# Autodesk Inventor assembly: GP5-100
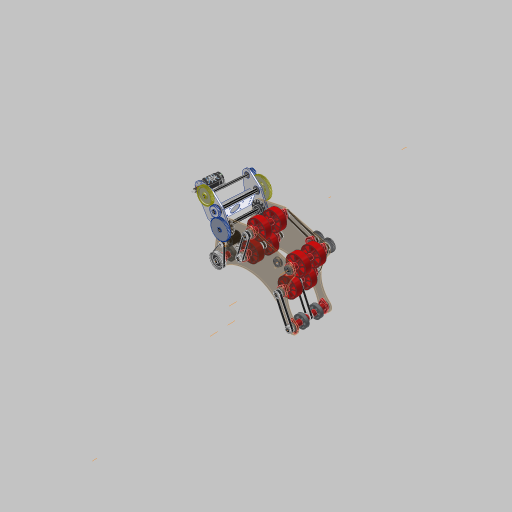
[picture p0: Inventor's stored thumbnail of the model, 512x512]
Saved by Autodesk Inventor 2023.5 (Build 275446000, 446)
## iProperties
Created: 2025-02-03
Part Number: GP5-100
Document SubType Name: Assembly
Designer: slick
Author: slick
## Documents named in this file (27)
- C:\Users\slick\OneDrive\Desktop\2025-ReefScape---CAD\Gripper\GP5\GP5-100.iam
- C:\Users\slick\OneDrive\Desktop\2025-ReefScape---CAD\Gripper\GP5\GP5-003.ipt
- C:\Users\slick\OneDrive\Desktop\2025-ReefScape---CAD\COMMON PARTS\BEARINGS\13_75mm_1_2_ThunderHex_ID_x_1_125_OD_x_0_313_WD_Flanged_Bearing_217-4006_MIR.ipt
- C:\Users\slick\OneDrive\Desktop\2025-ReefScape---CAD\Gripper\GP5\GP5-005.ipt
- C:\Users\slick\OneDrive\Desktop\2025-ReefScape---CAD\COMMON PARTS\WHEELS\2_OD_Straight_Flex_Wheel_217-6354.ipt
- C:\Users\slick\OneDrive\Desktop\2025-ReefScape---CAD\COMMON PARTS\WHEELS\am-3946 3IN 375Hex Compliant Wheel REV 3.ipt
- C:\Users\slick\OneDrive\Desktop\2025-ReefScape---CAD\COMMON PARTS\MOTORS\Minion.ipt
- C:\Users\slick\OneDrive\Desktop\2025-ReefScape---CAD\COMMON PARTS\PULLEYS\gt2\16T Gt2 Kracken PullyWCP-1178.ipt
- C:\Users\slick\OneDrive\Desktop\2025-ReefScape---CAD\COMMON PARTS\PULLEYS\gt2\60t_x_9mm_Wide_Double_Flange_Aluminum_Pulley_GT2_3mm_1_2_Hex_Bore_217-5876.ipt
- C:\Users\slick\OneDrive\Desktop\2025-ReefScape---CAD\COMMON PARTS\PULLEYS\gt2\24t_x_9mm_Wide_Double_Flange_Aluminum_Pulley_GT2_3mm_1_2_Hex_Bore_217-5875.ipt
- C:\Users\slick\OneDrive\Desktop\2025-ReefScape---CAD\COMMON PARTS\GEARS\20dp .5 hex\34t_Aluminum_Spur_Gear_20_DP_1_2_Hex_Bore_217-2706.ipt
- C:\Users\slick\OneDrive\Desktop\2025-ReefScape---CAD\Gripper\GP5\GP5-006.ipt
- C:\Users\slick\OneDrive\Desktop\2025-ReefScape---CAD\Gripper\GP5\GP5-007.ipt
- C:\Users\slick\OneDrive\Desktop\2025-ReefScape---CAD\Gripper\GP5\GP5-200.iam
- C:\Users\slick\OneDrive\Desktop\2025-ReefScape---CAD\COMMON PARTS\BEARINGS\Bearing Retainer\Retainer.ipt
- C:\Users\slick\OneDrive\Desktop\2025-ReefScape---CAD\Gripper\GP5\GT2-100T.ipt
- C:\Users\slick\OneDrive\Desktop\2025-ReefScape---CAD\Gripper\GP5\GT2-90T.ipt
- C:\Users\slick\OneDrive\Desktop\2025-ReefScape---CAD\Gripper\GP5\GT2-90T16-60.ipt
- C:\Users\slick\OneDrive\Desktop\2025-ReefScape---CAD\Gripper\GP5\GT2-105T.ipt
- C:\Users\slick\OneDrive\Desktop\2025-ReefScape---CAD\Gripper\GP5\GP5-013.ipt
- C:\Users\slick\OneDrive\Desktop\2025-ReefScape---CAD\Gripper\GP5\GP5-014.ipt
- C:\Users\slick\OneDrive\Desktop\2025-ReefScape---CAD\Gripper\GP5\GP5-015.ipt
- C:\Users\slick\OneDrive\Desktop\2025-ReefScape---CAD\Gripper\GP5\GP5-016.ipt
- C:\Users\slick\OneDrive\Desktop\2025-ReefScape---CAD\Gripper\GP5\GP5-017.ipt
- C:\Users\slick\OneDrive\Desktop\2025-ReefScape---CAD\Gripper\GP5\GP5-018.ipt
- C:\Users\slick\OneDrive\Desktop\2025-ReefScape---CAD\Gripper\GP5\GP5-019.ipt
- C:\Users\slick\OneDrive\Desktop\2025-ReefScape---CAD\COMMON PARTS\HUBS\WCP-1388.ipt
## Components (102 placed, 26 different names)
1. GP5-003:1 — Mate:7, Mate:9, Insert:12, Insert:13, Insert:14, Insert:15, Insert:16, Insert:17, Insert:18, Mate:49, Mate:59, Insert:21, Mate:64, Insert:22, Insert:23, Insert:24, Insert:25, Insert:26, Insert:27, Insert:28, Insert:29, Insert:30, Insert:31, Insert:32, Insert:33, Insert:34, Insert:35, Mate:137, Insert:49
2. GP5-003:2 — Mate:7, Mate:9, Insert:5, Insert:6, Insert:7, Insert:8, Insert:9, Insert:10, Insert:11, Mate:40, Mate:43, Mate:44, Insert:19, Mate:47, Mate:63, Insert:20, Insert:36, Insert:37, Insert:38, Insert:39, Insert:40, Insert:41, Insert:42, Insert:43, Insert:44, Insert:45, Insert:46, Insert:47, Mate:136, Insert:48
3. 13_75mm_1_2_ThunderHex_ID_x_1_125_OD_x_0_313_WD_Flanged_Bearing_217-4006_MIR:1 — Insert:5, Mate:20, Mate:46
4. 13_75mm_1_2_ThunderHex_ID_x_1_125_OD_x_0_313_WD_Flanged_Bearing_217-4006_MIR:2 — Insert:7, Mate:22
5. 13_75mm_1_2_ThunderHex_ID_x_1_125_OD_x_0_313_WD_Flanged_Bearing_217-4006_MIR:3 — Insert:6, Mate:21
6. 13_75mm_1_2_ThunderHex_ID_x_1_125_OD_x_0_313_WD_Flanged_Bearing_217-4006_MIR:4 — Insert:10, Mate:23, Mate:35, Mate:94
7. 13_75mm_1_2_ThunderHex_ID_x_1_125_OD_x_0_313_WD_Flanged_Bearing_217-4006_MIR:5 — Insert:9
8. 13_75mm_1_2_ThunderHex_ID_x_1_125_OD_x_0_313_WD_Flanged_Bearing_217-4006_MIR:6 — Insert:11, Mate:25
9. 13_75mm_1_2_ThunderHex_ID_x_1_125_OD_x_0_313_WD_Flanged_Bearing_217-4006_MIR:7 — Insert:8, Mate:24
10. 13_75mm_1_2_ThunderHex_ID_x_1_125_OD_x_0_313_WD_Flanged_Bearing_217-4006_MIR:8 — Insert:12
11. 13_75mm_1_2_ThunderHex_ID_x_1_125_OD_x_0_313_WD_Flanged_Bearing_217-4006_MIR:9 — Insert:15
12. 13_75mm_1_2_ThunderHex_ID_x_1_125_OD_x_0_313_WD_Flanged_Bearing_217-4006_MIR:10 — Insert:14
13. 13_75mm_1_2_ThunderHex_ID_x_1_125_OD_x_0_313_WD_Flanged_Bearing_217-4006_MIR:11 — Insert:16, Mate:54
14. 13_75mm_1_2_ThunderHex_ID_x_1_125_OD_x_0_313_WD_Flanged_Bearing_217-4006_MIR:12 — Insert:17
15. 13_75mm_1_2_ThunderHex_ID_x_1_125_OD_x_0_313_WD_Flanged_Bearing_217-4006_MIR:13 — Insert:13
16. 13_75mm_1_2_ThunderHex_ID_x_1_125_OD_x_0_313_WD_Flanged_Bearing_217-4006_MIR:14 — Insert:18
17. GP5-007:1 — Mate:25, Mate:28, Mate:62, Flush:26, Mate:65, Mate:67, Mate:89, Mate:112, Mate:113, Mate:128, Mate:129
18. GP5-006:1 — Mate:23, Mate:56, Flush:22, Mate:58, Mate:86, Mate:102, Mate:122
19. GP5-005:3 — Mate:24, Mate:34, Mate:60, Flush:25, Flush:27, Mate:66, Mate:68, Mate:87, Mate:88, Mate:93, Mate:103, Mate:124, Mate:126
20. GP5-005:4 — Mate:21, Mate:39, Mate:50, Flush:15, Mate:51, Flush:16, Mate:71, Mate:72, Mate:74, Mate:76, Mate:82, Mate:85, Mate:96, Mate:100, Mate:109
21. GP5-005:5 — Mate:22, Mate:38, Mate:52, Flush:17, Mate:53, Flush:18, Mate:84, Mate:90, Mate:95, Mate:101, Mate:120
22. GP5-005:6 — Mate:20, Mate:29, Flush:13, Mate:48, Mate:69, Mate:70, Mate:75, Mate:81, Mate:83, Mate:108, Mate:116, Mate:117, Mate:132, Mate:133
23. Minion:1 — Mate:43, Mate:44, Insert:19, Mate:45, Flush:12, Mate:80
24. 16T Gt2 Kracken PullyWCP-1178:1 — Mate:45, Flush:12
25. 60t_x_9mm_Wide_Double_Flange_Aluminum_Pulley_GT2_3mm_1_2_Hex_Bore_217-5876:1 — Mate:46, Flush:13, Mate:47, Flush:34
26. 24t_x_9mm_Wide_Double_Flange_Aluminum_Pulley_GT2_3mm_1_2_Hex_Bore_217-5875:1 — Mate:48, Mate:49, Flush:14, Mate:73
27. 24t_x_9mm_Wide_Double_Flange_Aluminum_Pulley_GT2_3mm_1_2_Hex_Bore_217-5875:2 — Mate:50, Flush:14, Flush:15, Flush:35
28. 24t_x_9mm_Wide_Double_Flange_Aluminum_Pulley_GT2_3mm_1_2_Hex_Bore_217-5875:3 — Mate:51, Flush:16, Flush:19, Flush:36
29. 24t_x_9mm_Wide_Double_Flange_Aluminum_Pulley_GT2_3mm_1_2_Hex_Bore_217-5875:4 — Mate:52, Flush:17, Flush:19
30. 24t_x_9mm_Wide_Double_Flange_Aluminum_Pulley_GT2_3mm_1_2_Hex_Bore_217-5875:5 — Mate:53, Flush:18, Flush:20, Flush:39
31. 24t_x_9mm_Wide_Double_Flange_Aluminum_Pulley_GT2_3mm_1_2_Hex_Bore_217-5875:6 — Mate:54, Flush:20, Mate:55, Mate:57, Mate:91
32. 34t_Aluminum_Spur_Gear_20_DP_1_2_Hex_Bore_217-2706:1 — Mate:55, Mate:57, Flush:21, Rotation:1
33. 34t_Aluminum_Spur_Gear_20_DP_1_2_Hex_Bore_217-2706:2 — Mate:56, Flush:21, Flush:22, Rotation:1
34. 24t_x_9mm_Wide_Double_Flange_Aluminum_Pulley_GT2_3mm_1_2_Hex_Bore_217-5875:7 — Mate:58, Mate:59, Flush:23
35. 24t_x_9mm_Wide_Double_Flange_Aluminum_Pulley_GT2_3mm_1_2_Hex_Bore_217-5875:8 — Mate:62, Flush:24, Flush:26, Flush:38
36. 24t_x_9mm_Wide_Double_Flange_Aluminum_Pulley_GT2_3mm_1_2_Hex_Bore_217-5875:9 — Mate:60, Mate:61, Flush:23, Flush:25, Flush:37
37. 24t_x_9mm_Wide_Double_Flange_Aluminum_Pulley_GT2_3mm_1_2_Hex_Bore_217-5875:10 — Mate:61, Mate:63, Flush:24, Flush:27
38. GP5-200:1 [sub-assembly] — Insert:20, Insert:21, Angle:1
39. Retainer:1 — Mate:64, Insert:22, Insert:23
40. Retainer:2 — Insert:24, Insert:25
41. Retainer:3 — Insert:26, Insert:27
42. Retainer:4 — Insert:28, Insert:29
43. Retainer:5 — Insert:30, Insert:31
44. Retainer:6 — Insert:32, Insert:33
45. Retainer:7 — Insert:34, Insert:35
46. Retainer:8 — Insert:36, Insert:37
47. Retainer:9 — Insert:38, Insert:39
48. Retainer:10 — Insert:46, Insert:47
49. Retainer:11 — Insert:40, Insert:41
50. Retainer:12 — Insert:42, Insert:43
51. Retainer:13 — Insert:44, Insert:45
52. GT2-100T:1 — Mate:73, Mate:74, Flush:31
53. GT2-100T:2 — Mate:75, Mate:76, Flush:30
54. GT2-100T:3 — Mate:65, Mate:66, Flush:29
55. 24t_x_9mm_Wide_Double_Flange_Aluminum_Pulley_GT2_3mm_1_2_Hex_Bore_217-5875:11 — Mate:67, Flush:28, Flush:29, Mate:130, Mate:131
56. 24t_x_9mm_Wide_Double_Flange_Aluminum_Pulley_GT2_3mm_1_2_Hex_Bore_217-5875:12 — Mate:68, Flush:28, Mate:79
57. 24t_x_9mm_Wide_Double_Flange_Aluminum_Pulley_GT2_3mm_1_2_Hex_Bore_217-5875:13 — Mate:69, Flush:32, Mate:77
58. 24t_x_9mm_Wide_Double_Flange_Aluminum_Pulley_GT2_3mm_1_2_Hex_Bore_217-5875:14 — Mate:70, Flush:33, Mate:77, Mate:111
59. 24t_x_9mm_Wide_Double_Flange_Aluminum_Pulley_GT2_3mm_1_2_Hex_Bore_217-5875:15 — Mate:71, Flush:30, Flush:33, Mate:110
60. 24t_x_9mm_Wide_Double_Flange_Aluminum_Pulley_GT2_3mm_1_2_Hex_Bore_217-5875:16 — Mate:72, Flush:31, Flush:32, Mate:78
61. GT2-90T16-60:1 — Mate:80, Mate:81, Flush:34
62. GT2-100T:4 — Flush:35, Mate:82, Mate:83
63. GT2-90T:1 — Mate:84, Mate:85, Flush:36
64. GT2-90T:2 — Mate:86, Mate:87, Flush:37
65. GT2-100T:5 — Mate:88, Mate:89, Flush:38
66. GT2-105T:1 — Mate:90, Flush:39, Mate:91
67. GP5-013:1 — Mate:95, Mate:98
68. GP5-013:2 — Mate:92, Mate:93
69. GP5-013:3 — Mate:96, Mate:97
70. GP5-013:4 — Mate:94, Mate:99
71. GP5-013:5 — Mate:101, Mate:107
72. GP5-013:6 — Mate:102, Mate:105
73. GP5-013:7 — Mate:100, Mate:106
74. GP5-013:8 — Mate:103, Mate:104
75. GP5-014:1 — Mate:108, Mate:111
76. GP5-014:2 — Mate:109, Mate:110
77. GP5-015:1 — Mate:116, Mate:119
78. GP5-015:2 — Mate:117, Mate:118
79. GP5-015:3 — Mate:112, Mate:115
80. GP5-015:4 — Mate:113, Mate:114
81. GP5-016:1 — Mate:122, Mate:123
82. GP5-016:2 — Mate:120, Mate:121
83. GP5-017:1 — Mate:124, Mate:125
84. GP5-017:2 — Mate:126, Mate:127
85. GP5-018:1 — Mate:128, Mate:131
86. GP5-018:2 — Mate:129, Mate:130
87. GP5-019:1 — Mate:133, Mate:134
88. GP5-019:2 — Mate:132, Mate:135
89. WCP-1388:1 — Mate:136, Insert:48
90. WCP-1388:2 — Mate:137, Insert:49, Angle:1
91. am-3946 3IN 375Hex Compliant Wheel REV 3:3 — Flush:7, Flush:9, Mate:33, Mate:40, Mate:97
92. am-3946 3IN 375Hex Compliant Wheel REV 3:2 — Flush:8, Flush:9, Mate:31, Mate:98, Mate:121
93. am-3946 3IN 375Hex Compliant Wheel REV 3:1 — Flush:8, Mate:30, Mate:37, Mate:99
94. am-3946 3IN 375Hex Compliant Wheel REV 3:4 — Flush:7, Mate:32, Mate:36, Mate:92, Mate:125
95. am-3946 3IN 375Hex Compliant Wheel REV 3:5 — Mate:78, Mate:106
96. am-3946 3IN 375Hex Compliant Wheel REV 3:6 — Mate:107
97. am-3946 3IN 375Hex Compliant Wheel REV 3:7 — Mate:105, Mate:123
98. am-3946 3IN 375Hex Compliant Wheel REV 3:8 — Flush:11, Mate:79, Mate:104, Mate:127
99. 2_OD_Straight_Flex_Wheel_217-6354:1 — Mate:27, Flush:10, Mate:118, Mate:135
100. 2_OD_Straight_Flex_Wheel_217-6354:2 — Mate:42, Flush:10, Mate:115
101. 2_OD_Straight_Flex_Wheel_217-6354:3 — Mate:119, Mate:134
102. 2_OD_Straight_Flex_Wheel_217-6354:4 — Flush:11, Mate:114
## Component patterns: (2 elements, first: am-3946 3IN 375Hex Compliant Wheel REV 3:3 + am-3946 3IN 375Hex Compliant Wheel REV 3:2 + am-3946 3IN 375Hex Compliant Wheel REV 3:1 + am-3946 3IN 375Hex Compliant Wheel REV 3:4), (2 elements, first: 2_OD_Straight_Flex_Wheel_217-6354:1 + 2_OD_Straight_Flex_Wheel_217-6354:2)
## Relationships (198: Mate 118, Insert 45, Flush 33, RelateRotation 1, Angle 1)
- Mate:7: GP5-003:1 ↔ GP5-003:2
- Mate:9: GP5-003:1 ↔ GP5-003:2
- Insert:5: GP5-003:2 ↔ 13_75mm_1_2_ThunderHex_ID_x_1_125_OD_x_0_313_WD_Flanged_Bearing_217-4006_MIR:1
- Insert:6: GP5-003:2 ↔ 13_75mm_1_2_ThunderHex_ID_x_1_125_OD_x_0_313_WD_Flanged_Bearing_217-4006_MIR:3
- Insert:7: GP5-003:2 ↔ 13_75mm_1_2_ThunderHex_ID_x_1_125_OD_x_0_313_WD_Flanged_Bearing_217-4006_MIR:2
- Insert:8: GP5-003:2 ↔ 13_75mm_1_2_ThunderHex_ID_x_1_125_OD_x_0_313_WD_Flanged_Bearing_217-4006_MIR:7
- Insert:9: GP5-003:2 ↔ 13_75mm_1_2_ThunderHex_ID_x_1_125_OD_x_0_313_WD_Flanged_Bearing_217-4006_MIR:5
- Insert:10: GP5-003:2 ↔ 13_75mm_1_2_ThunderHex_ID_x_1_125_OD_x_0_313_WD_Flanged_Bearing_217-4006_MIR:4
- Insert:11: GP5-003:2 ↔ 13_75mm_1_2_ThunderHex_ID_x_1_125_OD_x_0_313_WD_Flanged_Bearing_217-4006_MIR:6
- Insert:12: GP5-003:1 ↔ 13_75mm_1_2_ThunderHex_ID_x_1_125_OD_x_0_313_WD_Flanged_Bearing_217-4006_MIR:8
- Mate:20: 13_75mm_1_2_ThunderHex_ID_x_1_125_OD_x_0_313_WD_Flanged_Bearing_217-4006_MIR:1 ↔ GP5-005:6
- Mate:21: 13_75mm_1_2_ThunderHex_ID_x_1_125_OD_x_0_313_WD_Flanged_Bearing_217-4006_MIR:3 ↔ GP5-005:4
- Mate:22: 13_75mm_1_2_ThunderHex_ID_x_1_125_OD_x_0_313_WD_Flanged_Bearing_217-4006_MIR:2 ↔ GP5-005:5
- Mate:23: 13_75mm_1_2_ThunderHex_ID_x_1_125_OD_x_0_313_WD_Flanged_Bearing_217-4006_MIR:4 ↔ GP5-006:1
- Mate:24: 13_75mm_1_2_ThunderHex_ID_x_1_125_OD_x_0_313_WD_Flanged_Bearing_217-4006_MIR:7 ↔ GP5-005:3
- Mate:25: 13_75mm_1_2_ThunderHex_ID_x_1_125_OD_x_0_313_WD_Flanged_Bearing_217-4006_MIR:6 ↔ GP5-007:1
- Mate:27: 2_OD_Straight_Flex_Wheel_217-6354:1
- Mate:28: GP5-007:1
- Mate:29: GP5-005:6
- Flush:7: am-3946 3IN 375Hex Compliant Wheel REV 3:3 ↔ am-3946 3IN 375Hex Compliant Wheel REV 3:4
- Flush:8: am-3946 3IN 375Hex Compliant Wheel REV 3:2 ↔ am-3946 3IN 375Hex Compliant Wheel REV 3:1
- Flush:9: am-3946 3IN 375Hex Compliant Wheel REV 3:3 ↔ am-3946 3IN 375Hex Compliant Wheel REV 3:2
- Mate:30: am-3946 3IN 375Hex Compliant Wheel REV 3:1
- Mate:31: am-3946 3IN 375Hex Compliant Wheel REV 3:2
- Mate:32: am-3946 3IN 375Hex Compliant Wheel REV 3:4
- Mate:33: am-3946 3IN 375Hex Compliant Wheel REV 3:3
- Mate:34: GP5-005:3
- Mate:35: 13_75mm_1_2_ThunderHex_ID_x_1_125_OD_x_0_313_WD_Flanged_Bearing_217-4006_MIR:4
- Mate:36: am-3946 3IN 375Hex Compliant Wheel REV 3:4
- Mate:37: am-3946 3IN 375Hex Compliant Wheel REV 3:1
- Mate:38: GP5-005:5
- Mate:39: GP5-005:4
- Mate:40 (25.4 mm): GP5-003:2 ↔ am-3946 3IN 375Hex Compliant Wheel REV 3:3
- Mate:42: 2_OD_Straight_Flex_Wheel_217-6354:2
- Flush:10: 2_OD_Straight_Flex_Wheel_217-6354:1 ↔ 2_OD_Straight_Flex_Wheel_217-6354:2
- Flush:11: am-3946 3IN 375Hex Compliant Wheel REV 3:8 ↔ 2_OD_Straight_Flex_Wheel_217-6354:4
- Insert:13: GP5-003:1 ↔ 13_75mm_1_2_ThunderHex_ID_x_1_125_OD_x_0_313_WD_Flanged_Bearing_217-4006_MIR:13
- Insert:14: GP5-003:1 ↔ 13_75mm_1_2_ThunderHex_ID_x_1_125_OD_x_0_313_WD_Flanged_Bearing_217-4006_MIR:10
- Insert:15: GP5-003:1 ↔ 13_75mm_1_2_ThunderHex_ID_x_1_125_OD_x_0_313_WD_Flanged_Bearing_217-4006_MIR:9
- Insert:16: GP5-003:1 ↔ 13_75mm_1_2_ThunderHex_ID_x_1_125_OD_x_0_313_WD_Flanged_Bearing_217-4006_MIR:11
- Insert:17: GP5-003:1 ↔ 13_75mm_1_2_ThunderHex_ID_x_1_125_OD_x_0_313_WD_Flanged_Bearing_217-4006_MIR:12
- Insert:18: GP5-003:1 ↔ 13_75mm_1_2_ThunderHex_ID_x_1_125_OD_x_0_313_WD_Flanged_Bearing_217-4006_MIR:14
- Mate:43: GP5-003:2 ↔ Minion:1
- Mate:44: GP5-003:2 ↔ Minion:1
- Insert:19: GP5-003:2 ↔ Minion:1
- Mate:45: Minion:1 ↔ 16T Gt2 Kracken PullyWCP-1178:1
- Flush:12: Minion:1 ↔ 16T Gt2 Kracken PullyWCP-1178:1
- Mate:46: 13_75mm_1_2_ThunderHex_ID_x_1_125_OD_x_0_313_WD_Flanged_Bearing_217-4006_MIR:1 ↔ 60t_x_9mm_Wide_Double_Flange_Aluminum_Pulley_GT2_3mm_1_2_Hex_Bore_217-5876:1
- Flush:13: GP5-005:6 ↔ 60t_x_9mm_Wide_Double_Flange_Aluminum_Pulley_GT2_3mm_1_2_Hex_Bore_217-5876:1
- Mate:47: GP5-003:2 ↔ 60t_x_9mm_Wide_Double_Flange_Aluminum_Pulley_GT2_3mm_1_2_Hex_Bore_217-5876:1
- Mate:48: GP5-005:6 ↔ 24t_x_9mm_Wide_Double_Flange_Aluminum_Pulley_GT2_3mm_1_2_Hex_Bore_217-5875:1
- Mate:49: GP5-003:1 ↔ 24t_x_9mm_Wide_Double_Flange_Aluminum_Pulley_GT2_3mm_1_2_Hex_Bore_217-5875:1
- Mate:50: GP5-005:4 ↔ 24t_x_9mm_Wide_Double_Flange_Aluminum_Pulley_GT2_3mm_1_2_Hex_Bore_217-5875:2
- Flush:14: 24t_x_9mm_Wide_Double_Flange_Aluminum_Pulley_GT2_3mm_1_2_Hex_Bore_217-5875:1 ↔ 24t_x_9mm_Wide_Double_Flange_Aluminum_Pulley_GT2_3mm_1_2_Hex_Bore_217-5875:2
- Flush:15: GP5-005:4 ↔ 24t_x_9mm_Wide_Double_Flange_Aluminum_Pulley_GT2_3mm_1_2_Hex_Bore_217-5875:2
- Mate:51: GP5-005:4 ↔ 24t_x_9mm_Wide_Double_Flange_Aluminum_Pulley_GT2_3mm_1_2_Hex_Bore_217-5875:3
- Flush:16: GP5-005:4 ↔ 24t_x_9mm_Wide_Double_Flange_Aluminum_Pulley_GT2_3mm_1_2_Hex_Bore_217-5875:3
- Mate:52: GP5-005:5 ↔ 24t_x_9mm_Wide_Double_Flange_Aluminum_Pulley_GT2_3mm_1_2_Hex_Bore_217-5875:4
- Flush:17: GP5-005:5 ↔ 24t_x_9mm_Wide_Double_Flange_Aluminum_Pulley_GT2_3mm_1_2_Hex_Bore_217-5875:4
- Mate:53: GP5-005:5 ↔ 24t_x_9mm_Wide_Double_Flange_Aluminum_Pulley_GT2_3mm_1_2_Hex_Bore_217-5875:5
- Flush:18: GP5-005:5 ↔ 24t_x_9mm_Wide_Double_Flange_Aluminum_Pulley_GT2_3mm_1_2_Hex_Bore_217-5875:5
- Flush:19: 24t_x_9mm_Wide_Double_Flange_Aluminum_Pulley_GT2_3mm_1_2_Hex_Bore_217-5875:3 ↔ 24t_x_9mm_Wide_Double_Flange_Aluminum_Pulley_GT2_3mm_1_2_Hex_Bore_217-5875:4
- Mate:54: 13_75mm_1_2_ThunderHex_ID_x_1_125_OD_x_0_313_WD_Flanged_Bearing_217-4006_MIR:11 ↔ 24t_x_9mm_Wide_Double_Flange_Aluminum_Pulley_GT2_3mm_1_2_Hex_Bore_217-5875:6
- Flush:20: 24t_x_9mm_Wide_Double_Flange_Aluminum_Pulley_GT2_3mm_1_2_Hex_Bore_217-5875:5 ↔ 24t_x_9mm_Wide_Double_Flange_Aluminum_Pulley_GT2_3mm_1_2_Hex_Bore_217-5875:6
- Mate:55: 24t_x_9mm_Wide_Double_Flange_Aluminum_Pulley_GT2_3mm_1_2_Hex_Bore_217-5875:6 ↔ 34t_Aluminum_Spur_Gear_20_DP_1_2_Hex_Bore_217-2706:1
- Mate:56: GP5-006:1 ↔ 34t_Aluminum_Spur_Gear_20_DP_1_2_Hex_Bore_217-2706:2
- Mate:57: 24t_x_9mm_Wide_Double_Flange_Aluminum_Pulley_GT2_3mm_1_2_Hex_Bore_217-5875:6 ↔ 34t_Aluminum_Spur_Gear_20_DP_1_2_Hex_Bore_217-2706:1
- Flush:21: 34t_Aluminum_Spur_Gear_20_DP_1_2_Hex_Bore_217-2706:1 ↔ 34t_Aluminum_Spur_Gear_20_DP_1_2_Hex_Bore_217-2706:2
- Flush:22: GP5-006:1 ↔ 34t_Aluminum_Spur_Gear_20_DP_1_2_Hex_Bore_217-2706:2
- Mate:58: GP5-006:1 ↔ 24t_x_9mm_Wide_Double_Flange_Aluminum_Pulley_GT2_3mm_1_2_Hex_Bore_217-5875:7
- Mate:59: GP5-003:1 ↔ 24t_x_9mm_Wide_Double_Flange_Aluminum_Pulley_GT2_3mm_1_2_Hex_Bore_217-5875:7
- Mate:60: GP5-005:3 ↔ 24t_x_9mm_Wide_Double_Flange_Aluminum_Pulley_GT2_3mm_1_2_Hex_Bore_217-5875:9
- Mate:61: 24t_x_9mm_Wide_Double_Flange_Aluminum_Pulley_GT2_3mm_1_2_Hex_Bore_217-5875:9 ↔ 24t_x_9mm_Wide_Double_Flange_Aluminum_Pulley_GT2_3mm_1_2_Hex_Bore_217-5875:10
- Mate:62: GP5-007:1 ↔ 24t_x_9mm_Wide_Double_Flange_Aluminum_Pulley_GT2_3mm_1_2_Hex_Bore_217-5875:8
- Flush:23: 24t_x_9mm_Wide_Double_Flange_Aluminum_Pulley_GT2_3mm_1_2_Hex_Bore_217-5875:7 ↔ 24t_x_9mm_Wide_Double_Flange_Aluminum_Pulley_GT2_3mm_1_2_Hex_Bore_217-5875:9
- Mate:63: GP5-003:2 ↔ 24t_x_9mm_Wide_Double_Flange_Aluminum_Pulley_GT2_3mm_1_2_Hex_Bore_217-5875:10
- Flush:24: 24t_x_9mm_Wide_Double_Flange_Aluminum_Pulley_GT2_3mm_1_2_Hex_Bore_217-5875:8 ↔ 24t_x_9mm_Wide_Double_Flange_Aluminum_Pulley_GT2_3mm_1_2_Hex_Bore_217-5875:10
- Flush:25: GP5-005:3 ↔ 24t_x_9mm_Wide_Double_Flange_Aluminum_Pulley_GT2_3mm_1_2_Hex_Bore_217-5875:9
- Flush:26: GP5-007:1 ↔ 24t_x_9mm_Wide_Double_Flange_Aluminum_Pulley_GT2_3mm_1_2_Hex_Bore_217-5875:8
- Flush:27: GP5-005:3 ↔ 24t_x_9mm_Wide_Double_Flange_Aluminum_Pulley_GT2_3mm_1_2_Hex_Bore_217-5875:10
- Insert:20: GP5-003:2 ↔ GP5-200:1
- Insert:21: GP5-003:1 ↔ GP5-200:1
- Mate:64: GP5-003:1 ↔ Retainer:1
- Insert:22: GP5-003:1 ↔ Retainer:1
- Insert:23: GP5-003:1 ↔ Retainer:1
- Insert:24: GP5-003:1 ↔ Retainer:2
- Insert:25: GP5-003:1 ↔ Retainer:2
- Insert:26: GP5-003:1 ↔ Retainer:3
- Insert:27: GP5-003:1 ↔ Retainer:3
- Insert:28: GP5-003:1 ↔ Retainer:4
- Insert:29: GP5-003:1 ↔ Retainer:4
- Insert:30: GP5-003:1 ↔ Retainer:5
- Insert:31: GP5-003:1 ↔ Retainer:5
- Insert:32: GP5-003:1 ↔ Retainer:6
- Insert:33: GP5-003:1 ↔ Retainer:6
- Insert:34: GP5-003:1 ↔ Retainer:7
- Insert:35: GP5-003:1 ↔ Retainer:7
- Insert:36: GP5-003:2 ↔ Retainer:8
- Insert:37: GP5-003:2 ↔ Retainer:8
- Insert:38: GP5-003:2 ↔ Retainer:9
- Insert:39: GP5-003:2 ↔ Retainer:9
- Insert:40: GP5-003:2 ↔ Retainer:11
- Insert:41: GP5-003:2 ↔ Retainer:11
- Insert:42: GP5-003:2 ↔ Retainer:12
- Insert:43: GP5-003:2 ↔ Retainer:12
- Insert:44: GP5-003:2 ↔ Retainer:13
- Insert:45: GP5-003:2 ↔ Retainer:13
- Insert:46: GP5-003:2 ↔ Retainer:10
- Insert:47: GP5-003:2 ↔ Retainer:10
- Mate:65: GP5-007:1 ↔ GT2-100T:3
- Mate:66 (0.0762 mm): GP5-005:3 ↔ GT2-100T:3
- Mate:67: GP5-007:1 ↔ 24t_x_9mm_Wide_Double_Flange_Aluminum_Pulley_GT2_3mm_1_2_Hex_Bore_217-5875:11
- Mate:68: GP5-005:3 ↔ 24t_x_9mm_Wide_Double_Flange_Aluminum_Pulley_GT2_3mm_1_2_Hex_Bore_217-5875:12
- Flush:28: 24t_x_9mm_Wide_Double_Flange_Aluminum_Pulley_GT2_3mm_1_2_Hex_Bore_217-5875:11 ↔ 24t_x_9mm_Wide_Double_Flange_Aluminum_Pulley_GT2_3mm_1_2_Hex_Bore_217-5875:12
- Flush:29: GT2-100T:3 ↔ 24t_x_9mm_Wide_Double_Flange_Aluminum_Pulley_GT2_3mm_1_2_Hex_Bore_217-5875:11
- Mate:69: GP5-005:6 ↔ 24t_x_9mm_Wide_Double_Flange_Aluminum_Pulley_GT2_3mm_1_2_Hex_Bore_217-5875:13
- Mate:70: GP5-005:6 ↔ 24t_x_9mm_Wide_Double_Flange_Aluminum_Pulley_GT2_3mm_1_2_Hex_Bore_217-5875:14
- Mate:71: GP5-005:4 ↔ 24t_x_9mm_Wide_Double_Flange_Aluminum_Pulley_GT2_3mm_1_2_Hex_Bore_217-5875:15
- Mate:72: GP5-005:4 ↔ 24t_x_9mm_Wide_Double_Flange_Aluminum_Pulley_GT2_3mm_1_2_Hex_Bore_217-5875:16
- Mate:73: 24t_x_9mm_Wide_Double_Flange_Aluminum_Pulley_GT2_3mm_1_2_Hex_Bore_217-5875:1 ↔ GT2-100T:1
- Mate:74 (0.0762 mm): GP5-005:4 ↔ GT2-100T:1
- Mate:75: GP5-005:6 ↔ GT2-100T:2
- Mate:76 (0.0762 mm): GP5-005:4 ↔ GT2-100T:2
- Flush:30: GT2-100T:2 ↔ 24t_x_9mm_Wide_Double_Flange_Aluminum_Pulley_GT2_3mm_1_2_Hex_Bore_217-5875:15
- Flush:31: GT2-100T:1 ↔ 24t_x_9mm_Wide_Double_Flange_Aluminum_Pulley_GT2_3mm_1_2_Hex_Bore_217-5875:16
- Flush:32: 24t_x_9mm_Wide_Double_Flange_Aluminum_Pulley_GT2_3mm_1_2_Hex_Bore_217-5875:13 ↔ 24t_x_9mm_Wide_Double_Flange_Aluminum_Pulley_GT2_3mm_1_2_Hex_Bore_217-5875:16
- Flush:33: 24t_x_9mm_Wide_Double_Flange_Aluminum_Pulley_GT2_3mm_1_2_Hex_Bore_217-5875:14 ↔ 24t_x_9mm_Wide_Double_Flange_Aluminum_Pulley_GT2_3mm_1_2_Hex_Bore_217-5875:15
- Mate:77 (3.175 mm): 24t_x_9mm_Wide_Double_Flange_Aluminum_Pulley_GT2_3mm_1_2_Hex_Bore_217-5875:13 ↔ 24t_x_9mm_Wide_Double_Flange_Aluminum_Pulley_GT2_3mm_1_2_Hex_Bore_217-5875:14
- Mate:78 (1.5875 mm): 24t_x_9mm_Wide_Double_Flange_Aluminum_Pulley_GT2_3mm_1_2_Hex_Bore_217-5875:16 ↔ am-3946 3IN 375Hex Compliant Wheel REV 3:5
- Mate:79 (11.1125 mm): 24t_x_9mm_Wide_Double_Flange_Aluminum_Pulley_GT2_3mm_1_2_Hex_Bore_217-5875:12 ↔ am-3946 3IN 375Hex Compliant Wheel REV 3:8
- Mate:80: Minion:1 ↔ GT2-90T16-60:1
- Mate:81 (0.0762 mm): GP5-005:6 ↔ GT2-90T16-60:1
- Flush:34: 60t_x_9mm_Wide_Double_Flange_Aluminum_Pulley_GT2_3mm_1_2_Hex_Bore_217-5876:1 ↔ GT2-90T16-60:1
- Flush:35: 24t_x_9mm_Wide_Double_Flange_Aluminum_Pulley_GT2_3mm_1_2_Hex_Bore_217-5875:2 ↔ GT2-100T:4
- Mate:82: GP5-005:4 ↔ GT2-100T:4
- Mate:83 (0.0762 mm): GP5-005:6 ↔ GT2-100T:4
- Rotation:1 [RelateRotation] (1 ul): 34t_Aluminum_Spur_Gear_20_DP_1_2_Hex_Bore_217-2706:1 ↔ 34t_Aluminum_Spur_Gear_20_DP_1_2_Hex_Bore_217-2706:2
- Mate:84: GP5-005:5 ↔ GT2-90T:1
- Mate:85 (0.0762 mm): GP5-005:4 ↔ GT2-90T:1
- Mate:86: GP5-006:1 ↔ GT2-90T:2
- Mate:87 (0.0762 mm): GP5-005:3 ↔ GT2-90T:2
- Flush:36: 24t_x_9mm_Wide_Double_Flange_Aluminum_Pulley_GT2_3mm_1_2_Hex_Bore_217-5875:3 ↔ GT2-90T:1
- Flush:37: 24t_x_9mm_Wide_Double_Flange_Aluminum_Pulley_GT2_3mm_1_2_Hex_Bore_217-5875:9 ↔ GT2-90T:2
- Mate:88: GP5-005:3 ↔ GT2-100T:5
- Mate:89 (0.0762 mm): GP5-007:1 ↔ GT2-100T:5
- Flush:38: 24t_x_9mm_Wide_Double_Flange_Aluminum_Pulley_GT2_3mm_1_2_Hex_Bore_217-5875:8 ↔ GT2-100T:5
- Mate:90: GP5-005:5 ↔ GT2-105T:1
- Flush:39: 24t_x_9mm_Wide_Double_Flange_Aluminum_Pulley_GT2_3mm_1_2_Hex_Bore_217-5875:5 ↔ GT2-105T:1
- Mate:91 (0.0762 mm): 24t_x_9mm_Wide_Double_Flange_Aluminum_Pulley_GT2_3mm_1_2_Hex_Bore_217-5875:6 ↔ GT2-105T:1
- Mate:92: GP5-013:2 ↔ am-3946 3IN 375Hex Compliant Wheel REV 3:4
- Mate:93: GP5-005:3 ↔ GP5-013:2
- Mate:94: 13_75mm_1_2_ThunderHex_ID_x_1_125_OD_x_0_313_WD_Flanged_Bearing_217-4006_MIR:4 ↔ GP5-013:4
- Mate:95: GP5-005:5 ↔ GP5-013:1
- Mate:96: GP5-005:4 ↔ GP5-013:3
- Mate:97: GP5-013:3 ↔ am-3946 3IN 375Hex Compliant Wheel REV 3:3
- Mate:98: GP5-013:1 ↔ am-3946 3IN 375Hex Compliant Wheel REV 3:2
- Mate:99: GP5-013:4 ↔ am-3946 3IN 375Hex Compliant Wheel REV 3:1
- Mate:100: GP5-005:4 ↔ GP5-013:7
- Mate:101: GP5-005:5 ↔ GP5-013:5
- Mate:102: GP5-006:1 ↔ GP5-013:6
- Mate:103: GP5-005:3 ↔ GP5-013:8
- Mate:104: GP5-013:8 ↔ am-3946 3IN 375Hex Compliant Wheel REV 3:8
- Mate:105: GP5-013:6 ↔ am-3946 3IN 375Hex Compliant Wheel REV 3:7
- Mate:106: GP5-013:7 ↔ am-3946 3IN 375Hex Compliant Wheel REV 3:5
- Mate:107: GP5-013:5 ↔ am-3946 3IN 375Hex Compliant Wheel REV 3:6
- Mate:108: GP5-005:6 ↔ GP5-014:1
- Mate:109: GP5-005:4 ↔ GP5-014:2
- Mate:110: 24t_x_9mm_Wide_Double_Flange_Aluminum_Pulley_GT2_3mm_1_2_Hex_Bore_217-5875:15 ↔ GP5-014:2
- Mate:111: 24t_x_9mm_Wide_Double_Flange_Aluminum_Pulley_GT2_3mm_1_2_Hex_Bore_217-5875:14 ↔ GP5-014:1
- Mate:112: GP5-007:1 ↔ GP5-015:3
- Mate:113: GP5-007:1 ↔ GP5-015:4
- Mate:114: GP5-015:4 ↔ 2_OD_Straight_Flex_Wheel_217-6354:4
- Mate:115: GP5-015:3 ↔ 2_OD_Straight_Flex_Wheel_217-6354:2
- Mate:116: GP5-005:6 ↔ GP5-015:1
- Mate:117: GP5-005:6 ↔ GP5-015:2
- Mate:118: GP5-015:2 ↔ 2_OD_Straight_Flex_Wheel_217-6354:1
- Mate:119: GP5-015:1 ↔ 2_OD_Straight_Flex_Wheel_217-6354:3
- Mate:120: GP5-005:5 ↔ GP5-016:2
- Mate:121: GP5-016:2 ↔ am-3946 3IN 375Hex Compliant Wheel REV 3:2
- Mate:122: GP5-006:1 ↔ GP5-016:1
- Mate:123: GP5-016:1 ↔ am-3946 3IN 375Hex Compliant Wheel REV 3:7
- Mate:124: GP5-005:3 ↔ GP5-017:1
- Mate:125: GP5-017:1 ↔ am-3946 3IN 375Hex Compliant Wheel REV 3:4
- Mate:126: GP5-005:3 ↔ GP5-017:2
- Mate:127: GP5-017:2 ↔ am-3946 3IN 375Hex Compliant Wheel REV 3:8
- Mate:128: GP5-007:1 ↔ GP5-018:1
- Mate:129: GP5-007:1 ↔ GP5-018:2
- Mate:130: 24t_x_9mm_Wide_Double_Flange_Aluminum_Pulley_GT2_3mm_1_2_Hex_Bore_217-5875:11 ↔ GP5-018:2
- Mate:131: 24t_x_9mm_Wide_Double_Flange_Aluminum_Pulley_GT2_3mm_1_2_Hex_Bore_217-5875:11 ↔ GP5-018:1
- Mate:132: GP5-005:6 ↔ GP5-019:2
- Mate:133: GP5-005:6 ↔ GP5-019:1
- Mate:134: GP5-019:1 ↔ 2_OD_Straight_Flex_Wheel_217-6354:3
- Mate:135: GP5-019:2 ↔ 2_OD_Straight_Flex_Wheel_217-6354:1
- Mate:136: GP5-003:2 ↔ WCP-1388:1
- Mate:137: GP5-003:1 ↔ WCP-1388:2
- Insert:48: GP5-003:2 ↔ WCP-1388:1
- Insert:49: GP5-003:1 ↔ WCP-1388:2
- Angle:1 (0 deg): GP5-200:1 ↔ WCP-1388:2
